# Autodesk Inventor assembly: Montagem Carretel
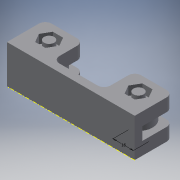
[picture p0: Inventor's stored thumbnail of the model, 180x180]
Saved by Autodesk Inventor 2017 (Build 210142000, 142)
## iProperties
Created: 2020-10-18
Part Number: Montagem Carretel
Document SubType Name: Assembly
Designer: ale
Author: ale
## Documents named in this file (4)
- C:\Users\ale\OneDrive\Pessoal\Eletrônica\Impressora 3D Core XY\Minha\Peças 3D\Montagem Carretel.iam
- C:\Users\ale\OneDrive\Pessoal\Eletrônica\Impressora 3D Core XY\Minha\Peças 3D\Suporte Carretel.ipt
- C:\Users\ale\OneDrive\Pessoal\Eletrônica\Impressora 3D Core XY\Minha\Peças 3D\rolamento.ipt
- C:\Users\ale\OneDrive\Pessoal\Eletrônica\Impressora 3D Core XY\Minha\Peças 3D\eixo.ipt
## Components (5 placed, 3 different names)
1. Suporte Carretel:1 — Flush:1, Mate:1, Insert:1, Insert:2
2. rolamento:1 — Insert:1
3. rolamento:2 — Insert:2
4. eixo:1 — Mate:1
5. eixo:2 — Flush:1
## Relationships (4: Insert 2, Flush 1, Mate 1)
- Flush:1: Suporte Carretel:1 ↔ eixo:2
- Mate:1: Suporte Carretel:1 ↔ eixo:1
- Insert:1 (2 mm): Suporte Carretel:1 ↔ rolamento:1
- Insert:2 (2 mm): Suporte Carretel:1 ↔ rolamento:2
